# Autodesk Inventor assembly: KS-15_all+air
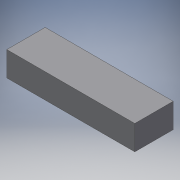
[picture p0: Inventor's stored thumbnail of the model, 180x180]
Saved by Autodesk Inventor 2018.2 (Build 222227000, 227)
## iProperties
Created: 2018-05-19
Part Number: KS-15_all+air
Material: 一般
Document SubType Name: Assembly
Designer: ku_sk
Author: ku_sk
## Documents named in this file (3)
- D:\ku_sk\ドキュメント\Inventor\Aero\KS-15\全体アッセンブリ解析用モデル\KS-15_all+air.iam
- D:\ku_sk\ドキュメント\Inventor\Aero\KS-15\全体アッセンブリ解析用モデル\air\air_Acceleration.ipt
- D:\ku_sk\ドキュメント\Inventor\Aero\KS-15\全体アッセンブリ解析用モデル\KS-15_all.iam
## Components (2 placed, 2 different names)
1. KS-15_all:1 [sub-assembly] — メイト:1, メイト:2, メイト:3, フラッシュ:1
2. air_Acceleration:1 — フラッシュ:1, フラッシュ:2
## Relationships (5: Mate 3, Flush 2)
- メイト:1 [Mate]: KS-15_all:1
- メイト:2 [Mate]: KS-15_all:1
- メイト:3 [Mate]: KS-15_all:1
- フラッシュ:1 [Flush] (-30 mm): KS-15_all:1 ↔ air_Acceleration:1
- フラッシュ:2 [Flush]: air_Acceleration:1
